# Autodesk Inventor assembly: joint_mag_assembly
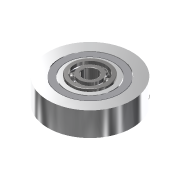
[picture p0: Inventor's stored thumbnail of the model, 180x180]
Saved by Autodesk Inventor 2017 (Build 210142000, 142)
## iProperties
Created: 2017-12-13
Part Number: joint_mag_assembly
Document SubType Name: Assembly
Designer: Thoma
Author: Thoma
## Documents named in this file (4)
- C:\Users\Thoma\Documents\SDUEmbedded\pendulum\joint\joint_mag_assembly.iam
- C:\Users\Thoma\Documents\master\components\joint\joint_mag_side.ipt
- C:\Users\Thoma\Documents\Inventor\Content Center Files\R2017\en-US\SKF 2Z - with two shields\SKF 2Z6201-2Z.ipt
- C:\Users\Thoma\Documents\master\components\joint\Axial rings\MR050C\MR050C.ipt
## Components (4 placed, 3 different names)
1. joint_mag_side:1 — Mate:1, Mate:2, Mate:3, Mate:5, Mate:6
2. SKF 2Z- with two shields SKF 2Z6201-2Z:1 — Mate:1, Mate:2, Mate:4
3. SKF 2Z- with two shields SKF 2Z6201-2Z:2 — Mate:3, Mate:4
4. MR050C:1 — Mate:5, Mate:6
## Relationships (6: Mate 6)
- Mate:1: joint_mag_side:1 ↔ SKF 2Z- with two shields SKF 2Z6201-2Z:1
- Mate:2: joint_mag_side:1 ↔ SKF 2Z- with two shields SKF 2Z6201-2Z:1
- Mate:3: joint_mag_side:1 ↔ SKF 2Z- with two shields SKF 2Z6201-2Z:2
- Mate:4: SKF 2Z- with two shields SKF 2Z6201-2Z:1 ↔ SKF 2Z- with two shields SKF 2Z6201-2Z:2
- Mate:5: joint_mag_side:1 ↔ MR050C:1
- Mate:6: joint_mag_side:1 ↔ MR050C:1
